# Autodesk Inventor assembly: X-Endstop
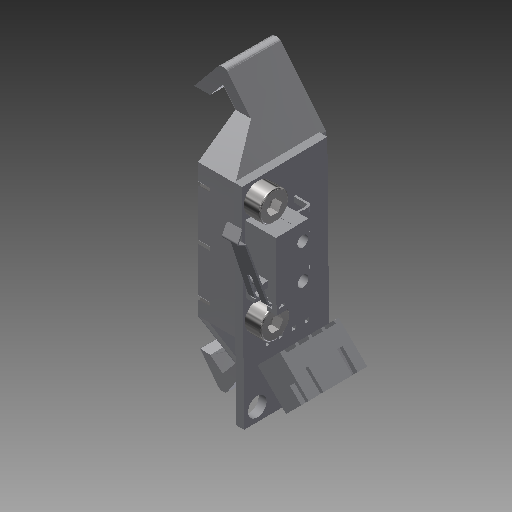
[picture p0: Inventor's stored thumbnail of the model, 512x512]
Saved by Autodesk Inventor 2017 (Build 210142000, 142)
## iProperties
Created: 2016-08-22
Part Number: X-Endstop
Document SubType Name: Assembly
Designer: User
Author: User
## Documents named in this file (5)
- C:\All INVENTOR\SL-Inventor\SL-Beast 3D Printer\X-Endstop.iam
- C:\All INVENTOR\SL-Inventor\SL-Beast 3D Printer\X Endstop Holder.ipt
- C:\All INVENTOR\SL-Inventor\SL-Beast 3D Printer\en-US\CSN EN 24 036\CSN EN 24 036 - M3.ipt
- C:\All INVENTOR\SL-Inventor\SL-Beast 3D Printer\Capteur fin de course.ipt
- C:\All INVENTOR\SL-Inventor\SL-Beast 3D Printer\en-US\ANSI B18.3.1M(6)\ANSI B18.3.1M - M3x0.5 x 10(1).ipt
## Components (6 placed, 4 different names)
1. X Endstop Holder:1
2. CSN EN 24036 M3:1
3. CSN EN 24036 M3:2
4. Capteur fin de course:1
5. Forged Socket Head Cap Screw - Metric M3x0.5 x 10:1
6. Forged Socket Head Cap Screw - Metric M3x0.5 x 10:2
## Relationships (10: Mate 8, Insert 2)
- [Mate]: X Endstop Holder:1 ↔ CSN EN 24036 M3:1
- [Mate]: X Endstop Holder:1 ↔ CSN EN 24036 M3:1
- [Mate]: X Endstop Holder:1 ↔ CSN EN 24036 M3:1
- [Mate]: X Endstop Holder:1 ↔ CSN EN 24036 M3:2
- [Mate]: X Endstop Holder:1 ↔ CSN EN 24036 M3:2
- [Mate]: X Endstop Holder:1 ↔ CSN EN 24036 M3:2
- [Mate]: X Endstop Holder:1 ↔ Capteur fin de course:1
- [Insert]: Capteur fin de course:1 ↔ Forged Socket Head Cap Screw - Metric M3x0.5 x 10:1
- [Insert]: Capteur fin de course:1 ↔ Forged Socket Head Cap Screw - Metric M3x0.5 x 10:2
- [Mate]: CSN EN 24036 M3:1 ↔ Forged Socket Head Cap Screw - Metric M3x0.5 x 10:1
